# Autodesk Inventor assembly: face
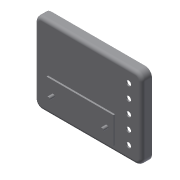
[picture p0: Inventor's stored thumbnail of the model, 180x180]
Saved by Autodesk Inventor 2022 (Build 260148000, 148)
## iProperties
Shininess: 64.0
Length Units: 11269
Angle Units: 11279
Time Units: 11290
Mass Units: 11283
Length Display Precision: 3
Angle Display Precision: 2
Created: 2002-04-17
Part Number: face
Document SubType Name: Assembly
Designer: Administrator
Density: 0.0
Volumn: 0.0
Area: 0.0
PropertySet Name: Model Information
Control State: 0
Master: False
Checked Out: False
Author: Administrator
## Documents named in this file (3)
- C:\Autodesk Inventor 2022 Advanced Assembly Modeling Practice Files\face.iam
- C:\Autodesk Inventor 2022 Advanced Assembly Modeling Practice Files\coverplate.ipt
- C:\Autodesk Inventor 2022 Advanced Assembly Modeling Practice Files\frontface.ipt
## Components (2 placed, 2 different names)
1. frontface:1 — Insert:1, Mate:1
2. coverplate:1 — Insert:1, Mate:1
## Relationships (2: Insert 1, Mate 1)
- Insert:1: frontface:1 ↔ coverplate:1
- Mate:1: frontface:1 ↔ coverplate:1
